# Autodesk Inventor assembly: Wing Left
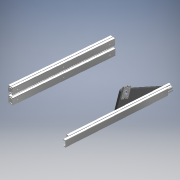
[picture p0: Inventor's stored thumbnail of the model, 180x180]
Saved by Autodesk Inventor 2019 (Build 230136000, 136)
## iProperties
Part Number: Wing Left
Document SubType Name: Assembly
Designer: Delta
Author: Delta
## Documents named in this file (4)
- C:\Robotics\CAD\2019-20_CAD\Collection\Wing Left.iam
- C:\Robotics\CAD\2019-20_CAD\Collection\Triangle axle slide connector.ipt
- C:\Robotics\CAD\COTSParts\Rev\REV-41-1683 Bear Blocks.ipt
- C:\Robotics\CAD\COTSParts\Misumi_Slides\AIS2018\SAR330.iam
## Components (5 placed, 3 different names)
1. Triangle axle slide connector:1 — Mate:3, Mate:4, Angle:1, Mate:5, Mate:6
2. REV-41-1683 Bear Blocks:1 — Mate:3, Mate:4, Angle:1
3. SAR330:1 [sub-assembly] — Mate:5, Mate:6
4. SAR330:2 [sub-assembly]
5. SAR330:3 [sub-assembly]
## Relationships (5: Mate 4, Angle 1)
- Mate:3: Triangle axle slide connector:1 ↔ REV-41-1683 Bear Blocks:1
- Mate:4: Triangle axle slide connector:1 ↔ REV-41-1683 Bear Blocks:1
- Angle:1 (0 deg): Triangle axle slide connector:1 ↔ REV-41-1683 Bear Blocks:1
- Mate:5: Triangle axle slide connector:1 ↔ SAR330:1
- Mate:6: Triangle axle slide connector:1 ↔ SAR330:1
